# Autodesk Inventor assembly: MG-Display mit Housing
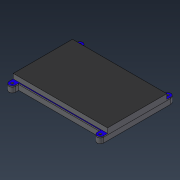
[picture p0: Inventor's stored thumbnail of the model, 180x180]
Saved by Autodesk Inventor 2022.3 (Build 263350000, 350)
## iProperties
Part Number: MG-Display mit Housing
Material: Generisch
Document SubType Name: Assembly
Designer: rYan
Author: rYan
## Documents named in this file (3)
- D:\TIGERsGIT\Hardware\mechanik\2020\Inventor\Tools\Display 5inch\MG-Display mit Housing.iam
- D:\TIGERsGIT\Hardware\mechanik\2020\Inventor\Tools\Display 5inch\Display 5inch Housing.ipt
- D:\TIGERsGIT\Hardware\mechanik\2020\Inventor\Purchased Parts\Display 5inch JRP5002.ipt
## Components (2 placed, 1 different names)
1. Display 5inch JRP5002:1 — Fluchtend:1, Fluchtend:2, Fluchtend:3, Einfügen:1, Passend:1
2. Display 5inch JRP5002:2 — Einfügen:1, Passend:1
## Relationships (5: Flush 3, Insert 1, Mate 1)
- Fluchtend:1 [Flush]: Display 5inch JRP5002:1
- Fluchtend:2 [Flush]: Display 5inch JRP5002:1
- Fluchtend:3 [Flush]: Display 5inch JRP5002:1
- Einfügen:1 [Insert]: Display 5inch JRP5002:1 ↔ Display 5inch JRP5002:2
- Passend:1 [Mate]: Display 5inch JRP5002:1 ↔ Display 5inch JRP5002:2
